# Autodesk Inventor assembly: module1
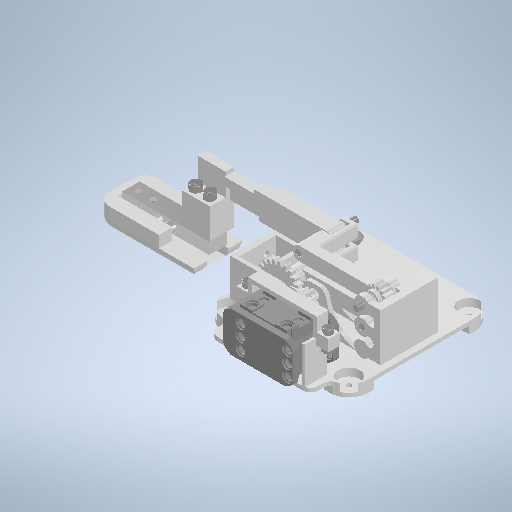
[picture p0: Inventor's stored thumbnail of the model, 512x512]
Saved by Autodesk Inventor 2025 (Build 290162000, 162)
## iProperties
Created: 2025-09-10
Part Number: module1
Document SubType Name: Assembly
Designer: sooo1
Author: sooo1
## Documents named in this file (33)
- C:\Users\sooo1\Downloads\final-20260216T060151Z-1-001\final\stroke_module\stroke_module.iam
- C:\Users\sooo1\Downloads\final-20260216T060151Z-1-001\final\stroke_module\link_arm2_1.iam
- C:\Users\sooo1\Downloads\final-20260216T060151Z-1-001\final\stroke_module\housing_shaft_linkl.ipt
- C:\Users\sooo1\Downloads\final-20260216T060151Z-1-001\final\stroke_module\shaft_Φ3_20.ipt
- C:\Users\sooo1\Downloads\final-20260216T060151Z-1-001\final\stroke_module\spacer_Φ3.2_1.ipt
- C:\Users\sooo1\Downloads\final-20260216T060151Z-1-001\final\stroke_module\shaft_Φ3_30.ipt
- C:\Users\sooo1\Downloads\final-20260216T060151Z-1-001\final\stroke_module\load_cell_SC616C.ipt
- C:\Users\sooo1\Downloads\final-20260216T060151Z-1-001\final\stroke_module\pressure_plate.ipt
- C:\Users\sooo1\Downloads\final-20260216T060151Z-1-001\final\stroke_module\link_arm_1_3.ipt
- C:\Users\sooo1\Downloads\final-20260216T060151Z-1-001\final\stroke_module\XL-320.ipt
- C:\Users\sooo1\Downloads\final-20260216T060151Z-1-001\final\stroke_module\shaft_Φ2_14.ipt
- C:\Users\sooo1\Downloads\final-20260216T060151Z-1-001\final\stroke_module\housing_xl320.ipt
- C:\Users\sooo1\Downloads\final-20260216T060151Z-1-001\final\stroke_module\link_arm_2.ipt
- C:\Users\sooo1\Downloads\final-20260216T060151Z-1-001\final\stroke_module\housing_shaft_link_base_4.ipt
- C:\Users\sooo1\Downloads\final-20260216T060151Z-1-001\final\stroke_module\spacer_Φ2.2_2.ipt
- C:\Users\sooo1\Downloads\final-20260216T060151Z-1-001\final\stroke_module\link_arm_5_2.ipt
- C:\Users\sooo1\Downloads\final-20260216T060151Z-1-001\final\stroke_module\housing_shaft_linkl_3.ipt
- C:\Users\sooo1\Downloads\final-20260216T060151Z-1-001\final\stroke_module\link_arm_6.ipt
- C:\Users\sooo1\Downloads\final-20260216T060151Z-1-001\final\stroke_module\housing_shaft_link_base_3.ipt
- C:\Users\sooo1\Downloads\final-20260216T060151Z-1-001\final\stroke_module\spacer_Φ3.2_13.ipt
- C:\Users\sooo1\Downloads\final-20260216T060151Z-1-001\final\stroke_module\spacer_Φ3.2_23.ipt
- C:\Users\sooo1\Downloads\final-20260216T060151Z-1-001\final\stroke_module\spacer_Φ3.2_20.ipt
- C:\Users\sooo1\Downloads\final-20260216T060151Z-1-001\final\stroke_module\gear_7.ipt
- C:\Users\sooo1\Downloads\final-20260216T060151Z-1-001\final\stroke_module\link_arm_b.ipt
- C:\Users\sooo1\Downloads\final-20260216T060151Z-1-001\final\stroke_module\spacer_Φ3.2_4_1.ipt
- C:\Users\sooo1\Downloads\final-20260216T060151Z-1-001\final\stroke_module\spacer_Φ3.2_5.ipt
- C:\Users\sooo1\Downloads\final-20260216T060151Z-1-001\final\stroke_module\link_arm2_p1.ipt
- C:\Users\sooo1\Downloads\final-20260216T060151Z-1-001\final\stroke_module\link_arm_p2.ipt
- C:\Users\sooo1\Downloads\final-20260216T060151Z-1-001\final\stroke_module\link_arm_1_2.ipt
- C:\Users\sooo1\Downloads\final-20260216T060151Z-1-001\final\stroke_module\JIS B 1181 - M2.5.ipt
- C:\Users\sooo1\Downloads\final-20260216T060151Z-1-001\final\stroke_module\JIS B 1176 - M3 x 20 - 0.5.ipt
- C:\Users\sooo1\Downloads\final-20260216T060151Z-1-001\final\stroke_module\JIS B 1176 - M3 x 10 - 0.5.ipt
- C:\Users\sooo1\Downloads\final-20260216T060151Z-1-001\final\stroke_module\JIS B 1176 - M2.5 x 8 - 0.45.ipt
## Components (61 placed, 32 different names)
1. JIS B 1181 上 等級 2 - メートル 等級 2 上 M2.5:1 — メイト:394, メイト:409
2. JIS B 1181 上 等級 2 - メートル 等級 2 上 M2.5:2 — メイト:396, メイト:410
3. JIS B 1176 - メートル M3 x 20:1 — メイト:399, メイト:400
4. JIS B 1176 - メートル M3 x 20:2 — メイト:397, メイト:398
5. JIS B 1176 - メートル M3 x 10:1 — メイト:402, メイト:404
6. JIS B 1176 - メートル M3 x 10:2 — メイト:401, メイト:403
7. JIS B 1176 - メートル M2.5 x 8:1 — メイト:405, メイト:408, メイト:409
8. JIS B 1176 - メートル M2.5 x 8:2 — メイト:406, メイト:407, メイト:410
9. spacer_Φ3.2_4_1:2 — メイト:357, メイト:358
10. spacer_Φ3.2_4_1:1 — メイト:355, メイト:356, メイト:359
11. link_arm_b:3 — メイト:350, メイト:351, メイト:352, 角度:9, 角度:10, メイト:369, メイト:373
12. gear_7:1 — メイト:347, メイト:348, メイト:349
13. spacer_Φ3.2_13:1 — メイト:335, メイト:351
14. shaft_Φ3_30:1 — メイト:235, メイト:253, フラッシュ:40, メイト:289
15. housing_shaft_link_base_4:1 — メイト:235, メイト:238, メイト:239, メイト:240, メイト:243, メイト:252, メイト:259, フラッシュ:40, メイト:280, フラッシュ:43, メイト:283, メイト:303, メイト:304, メイト:344, フラッシュ:57, メイト:345, フラッシュ:58, 角度:10, メイト:394, メイト:396
16. XL-320:2 — メイト:238, メイト:239, メイト:240, メイト:241, メイト:242, メイト:250, メイト:347, メイト:348, メイト:349
17. housing_xl320:2 — メイト:241, メイト:242, メイト:243, メイト:405, メイト:406, メイト:407, メイト:408
18. shaft_Φ3_30:2 — メイト:280, フラッシュ:43, メイト:282, メイト:335, メイト:350
19. spacer_Φ3.2_1:17 — メイト:282, メイト:283, メイト:369
20. spacer_Φ3.2_1:15 — メイト:248, メイト:253, メイト:259
21. link_arm_6:1 — メイト:271, メイト:292, メイト:299, フラッシュ:45, 角度:12, メイト:370, メイト:371, 角度:13
22. link_arm_5_2:1 — メイト:271, メイト:277, メイト:291, メイト:292, メイト:296, メイト:297, メイト:298, メイト:397, メイト:398, メイト:399, メイト:400
23. load_cell_SC616C:2 — メイト:296, メイト:297, メイト:298, メイト:355, メイト:356, メイト:357, メイト:358, メイト:401, メイト:402
24. pressure_plate:2 — メイト:359, メイト:403, メイト:404
25. shaft_Φ3_30:3 — メイト:299, フラッシュ:45
26. housing_shaft_linkl_3:1 — メイト:370, メイト:371, メイト:372, メイト:373, フラッシュ:59, メイト:374, フラッシュ:60, メイト:375, フラッシュ:61
27. shaft_Φ3_20:8 — メイト:352, フラッシュ:59
28. shaft_Φ3_20:9 — メイト:374, フラッシュ:60
29. shaft_Φ3_30:4 — メイト:375, フラッシュ:61
30. link_arm_2:1 — メイト:248, メイト:279, メイト:289, メイト:354, 角度:12
31. link_arm2_1:2 [sub-assembly] — メイト:276, メイト:277, フラッシュ:41, メイト:279, 角度:9, メイト:354, 角度:13, メイト:372
32. shaft_Φ3_20:7 — メイト:276, フラッシュ:41, メイト:291
33. shaft_Φ2_14:2 — メイト:250, メイト:251
34. spacer_Φ2.2_2:1 — メイト:251, メイト:252
35. JIS B 1176 - メートル M3 x 20:3 — メイト:411, メイト:413
36. JIS B 1176 - メートル M3 x 20:4 — メイト:412, メイト:414
37. JIS B 1176 - メートル M3 x 10:3 — メイト:416, メイト:417
38. JIS B 1176 - メートル M3 x 10:4 — メイト:415, メイト:418
39. link_arm_1_2:1 — メイト:385, メイト:386, メイト:387, 角度:15, メイト:388
40. link_arm_p2:1 — メイト:379, メイト:380, メイト:381, メイト:382
41. link_arm2_p1:1 — メイト:376, メイト:377, メイト:378, 角度:14, メイト:383, メイト:384, 角度:15
42. spacer_Φ3.2_4_1:4 — メイト:365, メイト:366, メイト:368
43. spacer_Φ3.2_4_1:3 — メイト:364, メイト:367
44. spacer_Φ3.2_5:1 — メイト:360, メイト:384, メイト:387
45. spacer_Φ3.2_5:2 — メイト:362, メイト:363, メイト:379, メイト:382
46. shaft_Φ3_30:7 — メイト:341, フラッシュ:56, メイト:360, メイト:376, メイト:386
47. spacer_Φ3.2_23:1 — メイト:337, メイト:338
48. spacer_Φ3.2_20:1 — メイト:339, メイト:340
49. shaft_Φ3_20:10 — メイト:333, フラッシュ:54
50. spacer_Φ3.2_1:19 — メイト:330, メイト:331, メイト:388
51. spacer_Φ3.2_1:18 — メイト:325, メイト:326, メイト:380
52. shaft_Φ3_30:6 — メイト:314, フラッシュ:50, メイト:325, メイト:337, メイト:381
53. shaft_Φ3_30:5 — メイト:315, フラッシュ:49, メイト:330, メイト:339, メイト:385
54. link_arm_1_3:1 — メイト:163, メイト:312, メイト:333, フラッシュ:54, メイト:363
55. shaft_Φ3_20:5 — メイト:163, メイト:321, フラッシュ:51, メイト:362
56. shaft_Φ3_20:1 — メイト:332, メイト:377
57. housing_shaft_linkl:1 — メイト:321, フラッシュ:51, メイト:341, フラッシュ:56, メイト:378
58. housing_shaft_link_base_3:1 — メイト:303, メイト:304, メイト:314, メイト:315, フラッシュ:49, フラッシュ:50, メイト:326, メイト:331, メイト:338, メイト:340, フラッシュ:58, 角度:14
59. pressure_plate:3 — メイト:368, メイト:415, メイト:416, メイト:417, メイト:418
60. load_cell_SC616C:3 — メイト:364, メイト:365, メイト:366, メイト:367
61. link_arm_5_2:2 — メイト:312, メイト:332, メイト:383, メイト:411, メイト:412, メイト:413, メイト:414
## Relationships (139: Mate 119, Flush 14, Angle 6)
- メイト:163 [Mate]: link_arm_1_3:1 ↔ shaft_Φ3_20:5
- メイト:235 [Mate]: shaft_Φ3_30:1 ↔ housing_shaft_link_base_4:1
- メイト:238 [Mate]: housing_shaft_link_base_4:1 ↔ XL-320:2
- メイト:239 [Mate]: housing_shaft_link_base_4:1 ↔ XL-320:2
- メイト:240 [Mate]: housing_shaft_link_base_4:1 ↔ XL-320:2
- メイト:241 [Mate]: XL-320:2 ↔ housing_xl320:2
- メイト:242 [Mate]: XL-320:2 ↔ housing_xl320:2
- メイト:243 [Mate]: housing_shaft_link_base_4:1 ↔ housing_xl320:2
- メイト:248 [Mate]: spacer_Φ3.2_1:15 ↔ link_arm_2:1
- メイト:250 [Mate]: XL-320:2 ↔ shaft_Φ2_14:2
- メイト:251 [Mate]: shaft_Φ2_14:2 ↔ spacer_Φ2.2_2:1
- メイト:252 [Mate]: housing_shaft_link_base_4:1 ↔ spacer_Φ2.2_2:1
- メイト:253 [Mate]: shaft_Φ3_30:1 ↔ spacer_Φ3.2_1:15
- メイト:259 [Mate]: housing_shaft_link_base_4:1 ↔ spacer_Φ3.2_1:15
- フラッシュ:40 [Flush]: shaft_Φ3_30:1 ↔ housing_shaft_link_base_4:1
- メイト:271 [Mate]: link_arm_6:1 ↔ link_arm_5_2:1
- メイト:276 [Mate]: link_arm2_1:2 ↔ shaft_Φ3_20:7
- メイト:277 [Mate]: link_arm_5_2:1 ↔ link_arm2_1:2
- フラッシュ:41 [Flush]: link_arm2_1:2 ↔ shaft_Φ3_20:7
- メイト:279 [Mate]: link_arm_2:1 ↔ link_arm2_1:2
- メイト:280 [Mate]: housing_shaft_link_base_4:1 ↔ shaft_Φ3_30:2
- フラッシュ:43 [Flush]: housing_shaft_link_base_4:1 ↔ shaft_Φ3_30:2
- メイト:282 [Mate]: shaft_Φ3_30:2 ↔ spacer_Φ3.2_1:17
- メイト:283 [Mate]: housing_shaft_link_base_4:1 ↔ spacer_Φ3.2_1:17
- メイト:289 [Mate]: shaft_Φ3_30:1 ↔ link_arm_2:1
- メイト:291 [Mate]: link_arm_5_2:1 ↔ shaft_Φ3_20:7
- メイト:292 [Mate]: link_arm_6:1 ↔ link_arm_5_2:1
- [Mate]: load_cell_SC616C:2 ↔ pressure_plate:2
- [Mate]: load_cell_SC616C:2 ↔ pressure_plate:2
- メイト:296 [Mate]: link_arm_5_2:1 ↔ load_cell_SC616C:2
- メイト:297 [Mate]: link_arm_5_2:1 ↔ load_cell_SC616C:2
- メイト:298 [Mate]: link_arm_5_2:1 ↔ load_cell_SC616C:2
- メイト:299 [Mate]: link_arm_6:1 ↔ shaft_Φ3_30:3
- フラッシュ:45 [Flush]: link_arm_6:1 ↔ shaft_Φ3_30:3
- メイト:303 [Mate]: housing_shaft_link_base_4:1 ↔ housing_shaft_link_base_3:1
- メイト:304 [Mate]: housing_shaft_link_base_4:1 ↔ housing_shaft_link_base_3:1
- [Mate]: pressure_plate:3 ↔ load_cell_SC616C:3
- [Mate]: pressure_plate:3 ↔ load_cell_SC616C:3
- [Mate]: load_cell_SC616C:3 ↔ link_arm_5_2:2
- [Mate]: load_cell_SC616C:3 ↔ link_arm_5_2:2
- [Mate]: load_cell_SC616C:3 ↔ link_arm_5_2:2
- メイト:312 [Mate]: link_arm_1_3:1 ↔ link_arm_5_2:2
- メイト:314 [Mate]: shaft_Φ3_30:6 ↔ housing_shaft_link_base_3:1
- メイト:315 [Mate]: shaft_Φ3_30:5 ↔ housing_shaft_link_base_3:1
- フラッシュ:49 [Flush]: shaft_Φ3_30:5 ↔ housing_shaft_link_base_3:1
- フラッシュ:50 [Flush]: shaft_Φ3_30:6 ↔ housing_shaft_link_base_3:1
- メイト:321 [Mate]: shaft_Φ3_20:5 ↔ housing_shaft_linkl:1
- フラッシュ:51 [Flush]: shaft_Φ3_20:5 ↔ housing_shaft_linkl:1
- メイト:325 [Mate]: spacer_Φ3.2_1:18 ↔ shaft_Φ3_30:6
- メイト:326 [Mate]: spacer_Φ3.2_1:18 ↔ housing_shaft_link_base_3:1
- メイト:330 [Mate]: spacer_Φ3.2_1:19 ↔ shaft_Φ3_30:5
- メイト:331 [Mate]: spacer_Φ3.2_1:19 ↔ housing_shaft_link_base_3:1
- メイト:332 [Mate]: shaft_Φ3_20:1 ↔ link_arm_5_2:2
- メイト:333 [Mate]: shaft_Φ3_20:10 ↔ link_arm_1_3:1
- フラッシュ:54 [Flush]: shaft_Φ3_20:10 ↔ link_arm_1_3:1
- メイト:335 [Mate]: spacer_Φ3.2_13:1 ↔ shaft_Φ3_30:2
- メイト:337 [Mate]: spacer_Φ3.2_23:1 ↔ shaft_Φ3_30:6
- メイト:338 [Mate]: spacer_Φ3.2_23:1 ↔ housing_shaft_link_base_3:1
- メイト:339 [Mate]: spacer_Φ3.2_20:1 ↔ shaft_Φ3_30:5
- メイト:340 [Mate]: spacer_Φ3.2_20:1 ↔ housing_shaft_link_base_3:1
- メイト:341 [Mate]: shaft_Φ3_30:7 ↔ housing_shaft_linkl:1
- フラッシュ:56 [Flush]: shaft_Φ3_30:7 ↔ housing_shaft_linkl:1
- メイト:344 [Mate]: housing_shaft_link_base_4:1
- フラッシュ:57 [Flush]: housing_shaft_link_base_4:1
- メイト:345 [Mate]: housing_shaft_link_base_4:1
- フラッシュ:58 [Flush]: housing_shaft_link_base_4:1 ↔ housing_shaft_link_base_3:1
- メイト:347 [Mate]: gear_7:1 ↔ XL-320:2
- メイト:348 [Mate]: gear_7:1 ↔ XL-320:2
- メイト:349 [Mate]: gear_7:1 ↔ XL-320:2
- メイト:350 [Mate]: link_arm_b:3 ↔ shaft_Φ3_30:2
- メイト:351 [Mate]: link_arm_b:3 ↔ spacer_Φ3.2_13:1
- メイト:352 [Mate]: link_arm_b:3 ↔ shaft_Φ3_20:8
- 角度:9 [Angle] (0 deg): link_arm_b:3 ↔ link_arm2_1:2
- メイト:354 [Mate]: link_arm_2:1 ↔ link_arm2_1:2
- 角度:10 [Angle] (0 deg): link_arm_b:3 ↔ housing_shaft_link_base_4:1
- メイト:355 [Mate]: spacer_Φ3.2_4_1:1 ↔ load_cell_SC616C:2
- メイト:356 [Mate]: spacer_Φ3.2_4_1:1 ↔ load_cell_SC616C:2
- メイト:357 [Mate]: spacer_Φ3.2_4_1:2 ↔ load_cell_SC616C:2
- メイト:358 [Mate]: spacer_Φ3.2_4_1:2 ↔ load_cell_SC616C:2
- メイト:359 [Mate]: spacer_Φ3.2_4_1:1 ↔ pressure_plate:2
- メイト:360 [Mate]: spacer_Φ3.2_5:1 ↔ shaft_Φ3_30:7
- メイト:362 [Mate]: spacer_Φ3.2_5:2 ↔ shaft_Φ3_20:5
- メイト:363 [Mate]: spacer_Φ3.2_5:2 ↔ link_arm_1_3:1
- メイト:364 [Mate]: spacer_Φ3.2_4_1:3 ↔ load_cell_SC616C:3
- メイト:365 [Mate]: spacer_Φ3.2_4_1:4 ↔ load_cell_SC616C:3
- メイト:366 [Mate]: spacer_Φ3.2_4_1:4 ↔ load_cell_SC616C:3
- メイト:367 [Mate]: spacer_Φ3.2_4_1:3 ↔ load_cell_SC616C:3
- メイト:368 [Mate]: spacer_Φ3.2_4_1:4 ↔ pressure_plate:3
- メイト:369 [Mate]: link_arm_b:3 ↔ spacer_Φ3.2_1:17
- 角度:12 [Angle] (0 deg): link_arm_6:1 ↔ link_arm_2:1
- メイト:370 [Mate]: link_arm_6:1 ↔ housing_shaft_linkl_3:1
- メイト:371 [Mate]: link_arm_6:1 ↔ housing_shaft_linkl_3:1
- 角度:13 [Angle] (0 deg): link_arm_6:1 ↔ link_arm2_1:2
- メイト:372 [Mate]: housing_shaft_linkl_3:1 ↔ link_arm2_1:2
- メイト:373 [Mate]: link_arm_b:3 ↔ housing_shaft_linkl_3:1
- フラッシュ:59 [Flush]: housing_shaft_linkl_3:1 ↔ shaft_Φ3_20:8
- メイト:374 [Mate]: housing_shaft_linkl_3:1 ↔ shaft_Φ3_20:9
- フラッシュ:60 [Flush]: housing_shaft_linkl_3:1 ↔ shaft_Φ3_20:9
- メイト:375 [Mate]: housing_shaft_linkl_3:1 ↔ shaft_Φ3_30:4
- フラッシュ:61 [Flush]: housing_shaft_linkl_3:1 ↔ shaft_Φ3_30:4
- メイト:376 [Mate]: link_arm2_p1:1 ↔ shaft_Φ3_30:7
- メイト:377 [Mate]: link_arm2_p1:1 ↔ shaft_Φ3_20:1
- メイト:378 [Mate]: link_arm2_p1:1 ↔ housing_shaft_linkl:1
- 角度:14 [Angle] (0 deg): link_arm2_p1:1 ↔ housing_shaft_link_base_3:1
- メイト:379 [Mate]: link_arm_p2:1 ↔ spacer_Φ3.2_5:2
- メイト:380 [Mate]: link_arm_p2:1 ↔ spacer_Φ3.2_1:18
- メイト:381 [Mate]: link_arm_p2:1 ↔ shaft_Φ3_30:6
- メイト:382 [Mate]: link_arm_p2:1 ↔ spacer_Φ3.2_5:2
- メイト:383 [Mate] (1 mm): link_arm2_p1:1 ↔ link_arm_5_2:2
- メイト:384 [Mate]: link_arm2_p1:1 ↔ spacer_Φ3.2_5:1
- メイト:385 [Mate]: link_arm_1_2:1 ↔ shaft_Φ3_30:5
- メイト:386 [Mate]: link_arm_1_2:1 ↔ shaft_Φ3_30:7
- メイト:387 [Mate]: link_arm_1_2:1 ↔ spacer_Φ3.2_5:1
- 角度:15 [Angle] (0 deg): link_arm_1_2:1 ↔ link_arm2_p1:1
- メイト:388 [Mate]: link_arm_1_2:1 ↔ spacer_Φ3.2_1:19
- メイト:394 [Mate]: JIS B 1181 上 等級 2 - メートル 等級 2 上 M2.5:1 ↔ housing_shaft_link_base_4:1
- メイト:396 [Mate]: JIS B 1181 上 等級 2 - メートル 等級 2 上 M2.5:2 ↔ housing_shaft_link_base_4:1
- メイト:397 [Mate]: JIS B 1176 - メートル M3 x 20:2 ↔ link_arm_5_2:1
- メイト:398 [Mate]: JIS B 1176 - メートル M3 x 20:2 ↔ link_arm_5_2:1
- メイト:399 [Mate]: JIS B 1176 - メートル M3 x 20:1 ↔ link_arm_5_2:1
- メイト:400 [Mate]: JIS B 1176 - メートル M3 x 20:1 ↔ link_arm_5_2:1
- メイト:401 [Mate]: JIS B 1176 - メートル M3 x 10:2 ↔ load_cell_SC616C:2
- メイト:402 [Mate]: JIS B 1176 - メートル M3 x 10:1 ↔ load_cell_SC616C:2
- メイト:403 [Mate]: JIS B 1176 - メートル M3 x 10:2 ↔ pressure_plate:2
- メイト:404 [Mate]: JIS B 1176 - メートル M3 x 10:1 ↔ pressure_plate:2
- メイト:405 [Mate]: JIS B 1176 - メートル M2.5 x 8:1 ↔ housing_xl320:2
- メイト:406 [Mate]: JIS B 1176 - メートル M2.5 x 8:2 ↔ housing_xl320:2
- メイト:407 [Mate]: JIS B 1176 - メートル M2.5 x 8:2 ↔ housing_xl320:2
- メイト:408 [Mate]: JIS B 1176 - メートル M2.5 x 8:1 ↔ housing_xl320:2
- メイト:409 [Mate]: JIS B 1181 上 等級 2 - メートル 等級 2 上 M2.5:1 ↔ JIS B 1176 - メートル M2.5 x 8:1
- メイト:410 [Mate]: JIS B 1181 上 等級 2 - メートル 等級 2 上 M2.5:2 ↔ JIS B 1176 - メートル M2.5 x 8:2
- メイト:411 [Mate]: JIS B 1176 - メートル M3 x 20:3 ↔ link_arm_5_2:2
- メイト:412 [Mate]: JIS B 1176 - メートル M3 x 20:4 ↔ link_arm_5_2:2
- メイト:413 [Mate]: JIS B 1176 - メートル M3 x 20:3 ↔ link_arm_5_2:2
- メイト:414 [Mate]: JIS B 1176 - メートル M3 x 20:4 ↔ link_arm_5_2:2
- メイト:415 [Mate]: JIS B 1176 - メートル M3 x 10:4 ↔ pressure_plate:3
- メイト:416 [Mate]: JIS B 1176 - メートル M3 x 10:3 ↔ pressure_plate:3
- メイト:417 [Mate]: JIS B 1176 - メートル M3 x 10:3 ↔ pressure_plate:3
- メイト:418 [Mate]: JIS B 1176 - メートル M3 x 10:4 ↔ pressure_plate:3
## Named parameters: d679_d370 = 0 mm, d680_d371 = 0 mm, d697_d679_d370 = 0 mm, d698_d680_d371 = 0 mm, d700_d682 = 0 mm, d701_d683 = 0 mm, d702_d684 = 0 mm
